# Autodesk Inventor assembly: backplane
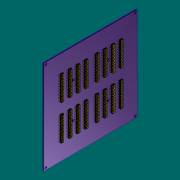
[picture p0: Inventor's stored thumbnail of the model, 180x180]
Saved by Autodesk Inventor 2016 (Build 200138000, 138)
## iProperties
Created: 2015-12-22
Part Number: backplane
Description: for SolidWorks
Document SubType Name: Assembly
Designer: sawai
Authority: Unknown
Sending System: Diptrace
Preprocessor: Open CASCADE STEP processor 6.6
Title: C:\Users\sawai\Desktop\backplane.step
Author: sawai
## Documents named in this file (3)
- C:\Users\sawaiz\oneDrive\projects\modularRICHBackplane\cad\backplane.iam
- C:\Users\sawaiz\oneDrive\projects\modularRICHBackplane\cad\backplane.ipt
- C:\Users\sawaiz\oneDrive\projects\modularRICHBackplane\cad\connectors\N182GFNS-RC.ipt
## Components (33 placed, 2 different names)
1. backplane:1 — Mate:1, Angle:1, Mate:2, Angle:2
2. N182GFNS-RC:1 — Mate:1, Angle:1
3. N182GFNS-RC:2
4. N182GFNS-RC:3
5. N182GFNS-RC:4
6. N182GFNS-RC:5
7. N182GFNS-RC:6
8. N182GFNS-RC:7
9. N182GFNS-RC:8
10. N182GFNS-RC:9
11. N182GFNS-RC:10
12. N182GFNS-RC:11
13. N182GFNS-RC:12
14. N182GFNS-RC:13
15. N182GFNS-RC:14
16. N182GFNS-RC:15
17. N182GFNS-RC:16
18. N182GFNS-RC:17 — Mate:2, Angle:2
19. N182GFNS-RC:18
20. N182GFNS-RC:19
21. N182GFNS-RC:20
22. N182GFNS-RC:21
23. N182GFNS-RC:22
24. N182GFNS-RC:23
25. N182GFNS-RC:24
26. N182GFNS-RC:25
27. N182GFNS-RC:26
28. N182GFNS-RC:27
29. N182GFNS-RC:28
30. N182GFNS-RC:29
31. N182GFNS-RC:30
32. N182GFNS-RC:31
33. N182GFNS-RC:32
## Component patterns: (4 elements), (4 elements), (4 elements, first: N182GFNS-RC:1), Component Pattern 3:2 (4 elements), Component Pattern 3:3 (4 elements), Component Pattern 3:4 (4 elements), (4 elements, first: N182GFNS-RC:17), Component Pattern 5:2 (4 elements), Component Pattern 5:3 (4 elements), Component Pattern 5:4 (4 elements)
## Relationships (4: Mate 2, Angle 2)
- Mate:1: backplane:1 ↔ N182GFNS-RC:1
- Angle:1 (0 deg): backplane:1 ↔ N182GFNS-RC:1
- Mate:2: backplane:1 ↔ N182GFNS-RC:17
- Angle:2 (0 deg): backplane:1 ↔ N182GFNS-RC:17
